# Autodesk Inventor assembly: arm simple 1
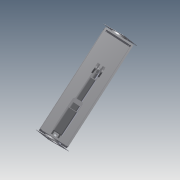
[picture p0: Inventor's stored thumbnail of the model, 180x180]
Saved by Autodesk Inventor 2011 (Build 150239000, 239)
## iProperties
Created: 2011-12-31
Part Number: arm simple 1
Document SubType Name: Assembly
Designer: Matthew
Author: Matthew
## Documents named in this file (9)
- C:\Users\Matthew\Documents\matthew_autocad\prlite\arm perhaps\ARM SIMPLE 1.iam
- C:\Users\Matthew\Documents\matthew_autocad\prlite\arm perhaps\1.ipt
- C:\Users\Matthew\Documents\matthew_autocad\prlite\arm perhaps\2.ipt
- C:\Users\Matthew\Documents\matthew_autocad\prlite\arm perhaps\tb2.ipt
- C:\Users\Matthew\Documents\matthew_autocad\prlite\arm perhaps\side.ipt
- C:\Users\Matthew\Documents\matthew_autocad\prlite\arm perhaps\back.ipt
- C:\Users\Matthew\Documents\matthew_autocad\prlite\arm perhaps\linacconnect.ipt
- C:\Users\Matthew\Documents\matthew_autocad\prlite\arm perhaps\linac body.ipt
- C:\Users\Matthew\Documents\matthew_autocad\prlite\arm perhaps\linac arm1.ipt
## Components (13 placed, 8 different names)
1. 1:1 — Mate:1, Mate:2, Mate:3, Mate:4, Mate:5
2. 2:1 — Mate:1, Mate:2, Flush:12
3. tb2:1 — Mate:3, Mate:4, Mate:5, Mate:6, Mate:7, Flush:2, Flush:3, Flush:4, Flush:5, Flush:6, Flush:7, Mate:18
4. side:1 — Mate:6, Flush:2, Flush:3, Flush:8, Mate:19
5. side:2 — Mate:7, Flush:4, Flush:5, Flush:9
6. back:1 — Flush:6, Flush:7, Mate:15, Mate:16, Mate:17, Mate:18
7. tb2:2 — Flush:8, Flush:9, Mate:10, Mate:11, Mate:12, Mate:19
8. 1:2 — Mate:10, Mate:11, Mate:12, Mate:13, Mate:14
9. 2:2 — Mate:13, Mate:14, Flush:12
10. linacconnect:1 — Mate:15, Mate:16, Mate:17, Mate:21, Mate:22
11. linacconnect:2 — Mate:23, Mate:24
12. linac body:1 — Mate:20, Flush:10, Flush:11, Mate:21, Mate:22
13. linac arm1:1 — Mate:20, Flush:10, Flush:11, Mate:23, Mate:24
## Relationships (33: Mate 22, Flush 11)
- Mate:1: 1:1 ↔ 2:1
- Mate:2: 1:1 ↔ 2:1
- Mate:3: 1:1 ↔ tb2:1
- Mate:4: 1:1 ↔ tb2:1
- Mate:5: 1:1 ↔ tb2:1
- Mate:6: tb2:1 ↔ side:1
- Mate:7: tb2:1 ↔ side:2
- Flush:2: tb2:1 ↔ side:1
- Flush:3: tb2:1 ↔ side:1
- Flush:4: tb2:1 ↔ side:2
- Flush:5: tb2:1 ↔ side:2
- Flush:6: tb2:1 ↔ back:1
- Flush:7: tb2:1 ↔ back:1
- Flush:8: side:1 ↔ tb2:2
- Flush:9: side:2 ↔ tb2:2
- Mate:10: tb2:2 ↔ 1:2
- Mate:11: tb2:2 ↔ 1:2
- Mate:12: tb2:2 ↔ 1:2
- Mate:13: 1:2 ↔ 2:2
- Mate:14: 1:2 ↔ 2:2
- Mate:15: back:1 ↔ linacconnect:1
- Mate:16: back:1 ↔ linacconnect:1
- Mate:17: back:1 ↔ linacconnect:1
- Mate:18: tb2:1 ↔ back:1
- Mate:19: side:1 ↔ tb2:2
- Mate:20: linac body:1 ↔ linac arm1:1
- Flush:10 (7.112 mm): linac body:1 ↔ linac arm1:1
- Flush:11: linac body:1 ↔ linac arm1:1
- Mate:21: linacconnect:1 ↔ linac body:1
- Mate:22 (1.11 mm): linacconnect:1 ↔ linac body:1
- Mate:23: linacconnect:2 ↔ linac arm1:1
- Mate:24 (3.65 mm): linacconnect:2 ↔ linac arm1:1
- Flush:12: 2:1 ↔ 2:2
